# Autodesk Inventor assembly: Antenna_unit_MIR
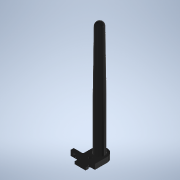
[picture p0: Inventor's stored thumbnail of the model, 180x180]
Saved by Autodesk Inventor 2020.4 (Build 244396000, 396)
## iProperties
Created: 2021-06-17
Part Number: Antenna_unit_MIR
Document SubType Name: Assembly
Designer: Masato Kubotera
Mass: 11.8411 g
Surface Area: 44.2768 cm^2
Volume: 8.30955 cm^3
Density: 1.425 g/cm^3
Author: Masato Kubotera
Title: Antenna_unit_MIR
## Documents named in this file (3)
- C:\Users\Masato\Documents\Inventor\CIT Brains_Inventor\OpenPlatform_ver3_0\UpperBody\Cockpit\Antenna_unit_MIR.iam
- C:\Users\Masato\Documents\Inventor\CIT Brains_Inventor\OpenPlatform_ver3_0\UpperBody\Cockpit\Antenna_frame_01_MIR.ipt
- C:\Users\Masato\Documents\Inventor\CIT Brains_Inventor\OpenPlatform_ver3_0\UpperBody\Cockpit\antenna.ipt
## Components (2 placed, 2 different names)
1. Antenna_frame_01_MIR:1 — 挿入:1
2. antenna:1 — 挿入:1
## Relationships (1: Insert 1)
- 挿入:1 [Insert]: Antenna_frame_01_MIR:1 ↔ antenna:1
